# Autodesk Inventor assembly: Diff_test
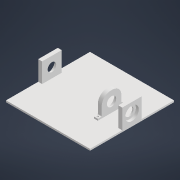
[picture p0: Inventor's stored thumbnail of the model, 180x180]
Saved by Autodesk Inventor 2021 (Build 250183000, 183)
## iProperties
Created: 2021-01-24
Part Number: Diff_test
Document SubType Name: Assembly
Designer: Ctroi
Author: Ctroi
## Documents named in this file (3)
- G:\Roverprojekt\Github Projekt\Rover\Diff_test.iam
- G:\Roverprojekt\Github Projekt\Rover\Testplatte_Differential.ipt
- G:\Roverprojekt\Github Projekt\Rover\Halterung_Differential.ipt
## Components (2 placed, 2 different names)
1. Testplatte_Differential:1 — Passend:1, Passend:2
2. Halterung_Differential:1 — Passend:1, Passend:2
## Relationships (2: Mate 2)
- Passend:1 [Mate]: Testplatte_Differential:1 ↔ Halterung_Differential:1
- Passend:2 [Mate]: Testplatte_Differential:1 ↔ Halterung_Differential:1
